# Autodesk Inventor assembly: PCBaseplateV2_CASLM_DecoupledBS
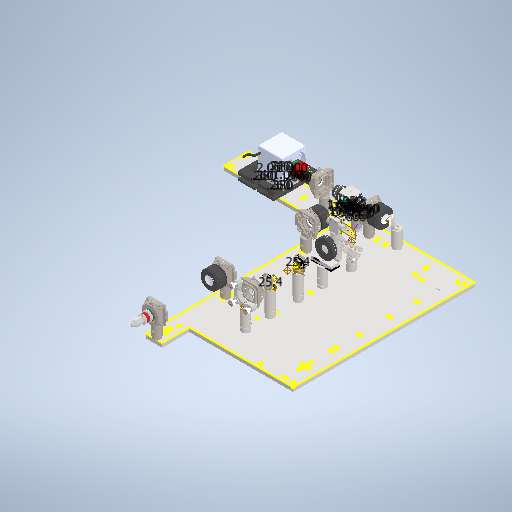
[picture p0: Inventor's stored thumbnail of the model, 512x512]
Saved by Autodesk Inventor 2025.2 (Build 292293000, 293)
## iProperties
Created: 2025-10-27
Part Number: PCBaseplateV2_CASLM_DecoupledBS
Document SubType Name: Assembly
Designer: monolithic
Author: monolithic
## Documents named in this file (17)
- C:\Users\monolithic\Documents\GitHub\CAD\Monolith\John\Altair_PowellAndCylindricalBaseplatesCombined_10_16_2025\Assemblies\C_ASLM\test\New folder\PCBaseplateV2_CASLM_DecoupledBS.iam
- C:\Users\monolithic\Documents\GitHub\CAD\Monolith\John\Altair_PowellAndCylindricalBaseplatesCombined_10_16_2025\Assemblies\C_ASLM\test\New folder\AC254-030-OnPost.iam
- C:\Users\monolithic\Documents\GitHub\CAD\Monolith\John\Altair_PowellAndCylindricalBaseplatesCombined_10_16_2025\Assemblies\C_ASLM\test\New folder\AC254-080-OnPost.iam
- C:\Users\monolithic\Documents\GitHub\CAD\Monolith\John\Altair_PowellAndCylindricalBaseplatesCombined_10_16_2025\Assemblies\C_ASLM\test\New folder\B1F-Mirror_OnPost.iam
- C:\Users\monolithic\Documents\GitHub\CAD\Monolith\John\Altair_PowellAndCylindricalBaseplatesCombined_10_16_2025\Assemblies\C_ASLM\test\New folder\Laser_OnPost.iam
- C:\Users\monolithic\Documents\GitHub\CAD\Monolith\John\Altair_PowellAndCylindricalBaseplatesCombined_10_16_2025\Assemblies\C_ASLM\test\New folder\TTL200-A-Mounted.iam
- C:\Users\monolithic\Documents\GitHub\CAD\Monolith\John\Altair_PowellAndCylindricalBaseplatesCombined_10_16_2025\Assemblies\C_ASLM\test\New folder\VoiceCoil_Assembly.iam
- C:\Users\monolithic\Documents\GitHub\CAD\Monolith\John\Altair_PowellAndCylindricalBaseplatesCombined_10_16_2025\Assemblies\C_ASLM\test\New folder\RFO-Mounted.iam
- C:\Users\monolithic\Documents\GitHub\CAD\Monolith\John\Altair_PowellAndCylindricalBaseplatesCombined_10_16_2025\Assemblies\C_ASLM\test\New folder\Cyl_Lens_OnPost.iam
- C:\Users\monolithic\Documents\GitHub\CAD\Monolith\John\Altair_PowellAndCylindricalBaseplatesCombined_10_16_2025\Assemblies\C_ASLM\test\New folder\ILO-Mounted.iam
- C:\Users\monolithic\Documents\GitHub\CAD\Monolith\John\Altair_PowellAndCylindricalBaseplatesCombined_10_16_2025\Assemblies\C_ASLM\test\New folder\BS_Assembly_Coupled_BSAdapterV9.iam
- C:\Users\monolithic\Documents\GitHub\CAD\Monolith\John\Altair_PowellAndCylindricalBaseplatesCombined_10_16_2025\Assemblies\C_ASLM\test\New folder\Atlair_PowellandCylindrical_Baseplate_V5.ipt
- C:\Users\monolithic\Documents\GitHub\CAD\Monolith\John\Altair_PowellBaseplate_SPIM_ASLM_CTASLM\Assembly\SubAssemblies\Galvo-Holder-PolarisMount_metal_v2.ipt
- C:\Users\monolithic\Documents\GitHub\CAD\Monolith\John\2026_2_9_CondensedCTASLMBaseplate\Assembly\Components\K1S4andMirrorNoPost.iam
- C:\Users\monolithic\Documents\GitHub\CAD\Monolith\John\Altair_PowellBaseplate_SPIM_ASLM_CTASLM\Assembly\SubAssemblies\Galvo_Galvo_Tilted.iam
- C:\Users\monolithic\Documents\GitHub\CAD\Monolith\John\PolarisPost_HeightAdjustment_0p77in_ForK1S4Mirrors_Machined.ipt
- C:\Users\monolithic\Documents\GitHub\CAD\Monolith\John\Altair_PowellAndCylindricalBaseplatesCombined_10_16_2025\Assemblies\C_ASLM\test\New folder\PLS-P3.ipt
## Components (18 placed, 16 different names)
1. AC254-030-OnPost:1 [sub-assembly] — Mate:59, Mate:76
2. AC254-080-OnPost:1 [sub-assembly] — Mate:60, Mate:77
3. B1F-Mirror_OnPost:1 [sub-assembly] — Mate:57, Mate:81
4. Laser_OnPost:1 [sub-assembly] — Mate:26, Mate:58
5. Atlair_PowellandCylindrical_Baseplate_V5:1 — Mate:26, Mate:34, Mate:37, Angle:8, Mate:39, Angle:9, Mate:51, Mate:52, Mate:57, Mate:58, Mate:59, Mate:60, Mate:62, Angle:15, Mate:63, Mate:68, Mate:70, Angle:18, Mate:71, Angle:19, Mate:73, Mate:75, Mate:76, Mate:77, Mate:78, Mate:81, Mate:82, Mate:83, Angle:20, Mate:84, Mate:86, Mate:87, Mate:88, Mate:91, Mate:92, Angle:22, Angle:23
6. TTL200-A-Mounted:1 [sub-assembly] — Mate:34, Mate:82
7. VoiceCoil_Assembly:1 [sub-assembly] — Mate:37, Angle:8, Mate:51
8. RFO-Mounted:1 [sub-assembly] — Mate:39, Angle:9, Mate:52
9. Cyl_Lens_OnPost:1 [sub-assembly] — Mate:62, Angle:15, Mate:78
10. TTL200-A-Mounted:2 [sub-assembly] — Mate:63, Mate:73
11. TTL200-A-Mounted:3 [sub-assembly] — Mate:68, Mate:70, Angle:18
12. ILO-Mounted:1 [sub-assembly] — Mate:71, Angle:19, Mate:75
13. BS_Assembly_Coupled_BSAdapterV9:1 [sub-assembly] — Mate:83, Angle:20, Mate:84
14. Galvo-Holder-PolarisMount_metal_v2:1 — Mate:93, Mate:94, Angle:23
15. K1S4andMirrorNoPost:1 [sub-assembly] — Mate:89, Mate:90
16. Galvo_Galvo_Tilted:1 [sub-assembly]
17. PolarisPost_HeightAdjustment_0p77in_ForK1S4Mirrors_Machined:1 — Mate:86, Mate:87, Mate:88, Mate:89, Mate:90
18. PLS-P3:1 — Mate:91, Mate:92, Angle:22, Mate:93, Mate:94
## Relationships (43: Mate 34, Angle 9)
- Mate:26: Laser_OnPost:1 ↔ Atlair_PowellandCylindrical_Baseplate_V5:1
- Mate:34: Atlair_PowellandCylindrical_Baseplate_V5:1 ↔ TTL200-A-Mounted:1
- Mate:37: Atlair_PowellandCylindrical_Baseplate_V5:1 ↔ VoiceCoil_Assembly:1
- Angle:8 (180 deg): Atlair_PowellandCylindrical_Baseplate_V5:1 ↔ VoiceCoil_Assembly:1
- Mate:39: Atlair_PowellandCylindrical_Baseplate_V5:1 ↔ RFO-Mounted:1
- Angle:9 (90 deg): Atlair_PowellandCylindrical_Baseplate_V5:1 ↔ RFO-Mounted:1
- Mate:51: Atlair_PowellandCylindrical_Baseplate_V5:1 ↔ VoiceCoil_Assembly:1
- Mate:52: Atlair_PowellandCylindrical_Baseplate_V5:1 ↔ RFO-Mounted:1
- Mate:57: B1F-Mirror_OnPost:1 ↔ Atlair_PowellandCylindrical_Baseplate_V5:1
- Mate:58: Laser_OnPost:1 ↔ Atlair_PowellandCylindrical_Baseplate_V5:1
- Mate:59: AC254-030-OnPost:1 ↔ Atlair_PowellandCylindrical_Baseplate_V5:1
- Mate:60: AC254-080-OnPost:1 ↔ Atlair_PowellandCylindrical_Baseplate_V5:1
- Mate:62: Atlair_PowellandCylindrical_Baseplate_V5:1 ↔ Cyl_Lens_OnPost:1
- Angle:15 (-90 deg): Atlair_PowellandCylindrical_Baseplate_V5:1 ↔ Cyl_Lens_OnPost:1
- Mate:63: Atlair_PowellandCylindrical_Baseplate_V5:1 ↔ TTL200-A-Mounted:2
- Mate:68: Atlair_PowellandCylindrical_Baseplate_V5:1 ↔ TTL200-A-Mounted:3
- Mate:70: Atlair_PowellandCylindrical_Baseplate_V5:1 ↔ TTL200-A-Mounted:3
- Angle:18 (90 deg): Atlair_PowellandCylindrical_Baseplate_V5:1 ↔ TTL200-A-Mounted:3
- Mate:71: Atlair_PowellandCylindrical_Baseplate_V5:1 ↔ ILO-Mounted:1
- Angle:19 (180 deg): Atlair_PowellandCylindrical_Baseplate_V5:1 ↔ ILO-Mounted:1
- Mate:73: Atlair_PowellandCylindrical_Baseplate_V5:1 ↔ TTL200-A-Mounted:2
- Mate:75: Atlair_PowellandCylindrical_Baseplate_V5:1 ↔ ILO-Mounted:1
- Mate:76: AC254-030-OnPost:1 ↔ Atlair_PowellandCylindrical_Baseplate_V5:1
- Mate:77: AC254-080-OnPost:1 ↔ Atlair_PowellandCylindrical_Baseplate_V5:1
- Mate:78: Atlair_PowellandCylindrical_Baseplate_V5:1 ↔ Cyl_Lens_OnPost:1
- Mate:81: B1F-Mirror_OnPost:1 ↔ Atlair_PowellandCylindrical_Baseplate_V5:1
- Mate:82: Atlair_PowellandCylindrical_Baseplate_V5:1 ↔ TTL200-A-Mounted:1
- Mate:83: Atlair_PowellandCylindrical_Baseplate_V5:1 ↔ BS_Assembly_Coupled_BSAdapterV9:1
- Angle:20 (0 deg): Atlair_PowellandCylindrical_Baseplate_V5:1 ↔ BS_Assembly_Coupled_BSAdapterV9:1
- Mate:84: Atlair_PowellandCylindrical_Baseplate_V5:1 ↔ BS_Assembly_Coupled_BSAdapterV9:1
- [Mate]: Galvo-Holder-PolarisMount_metal_v2:1 ↔ Galvo_Galvo_Tilted:1
- [Angle] (135 deg): Galvo-Holder-PolarisMount_metal_v2:1 ↔ Galvo_Galvo_Tilted:1
- Mate:86: Atlair_PowellandCylindrical_Baseplate_V5:1 ↔ PolarisPost_HeightAdjustment_0p77in_ForK1S4Mirrors_Machined:1
- Mate:87: Atlair_PowellandCylindrical_Baseplate_V5:1 ↔ PolarisPost_HeightAdjustment_0p77in_ForK1S4Mirrors_Machined:1
- Mate:88: Atlair_PowellandCylindrical_Baseplate_V5:1 ↔ PolarisPost_HeightAdjustment_0p77in_ForK1S4Mirrors_Machined:1
- Mate:89: K1S4andMirrorNoPost:1 ↔ PolarisPost_HeightAdjustment_0p77in_ForK1S4Mirrors_Machined:1
- Mate:90: K1S4andMirrorNoPost:1 ↔ PolarisPost_HeightAdjustment_0p77in_ForK1S4Mirrors_Machined:1
- Mate:91: Atlair_PowellandCylindrical_Baseplate_V5:1 ↔ PLS-P3:1
- Mate:92: Atlair_PowellandCylindrical_Baseplate_V5:1 ↔ PLS-P3:1
- Angle:22 (90 deg): Atlair_PowellandCylindrical_Baseplate_V5:1 ↔ PLS-P3:1
- Mate:93: Galvo-Holder-PolarisMount_metal_v2:1 ↔ PLS-P3:1
- Mate:94: Galvo-Holder-PolarisMount_metal_v2:1 ↔ PLS-P3:1
- Angle:23 (90 deg): Atlair_PowellandCylindrical_Baseplate_V5:1 ↔ Galvo-Holder-PolarisMount_metal_v2:1
